# Autodesk Inventor assembly: Stewart-Body-KST215MG
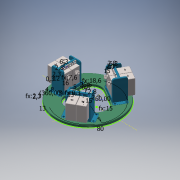
[picture p0: Inventor's stored thumbnail of the model, 180x180]
Saved by Autodesk Inventor 2018.2 (Build 222227000, 227)
## iProperties
Created: 2018-02-25
Part Number: Stewart-Body-KST215MG
Material: Generisch
Document SubType Name: Assembly
Designer: JochenAlt
Author: JochenAlt
## Documents named in this file (6)
- D:\Projects\Donna\CAD\KST DS215MG\Stewart-Body-KST215MG.iam
- D:\Projects\Donna\CAD\KST DS215MG\Stewart-Body.ipt
- D:\Projects\Donna\CAD\KST DS215MG\Stewart-Body-Servo-Holder-KST-DS215.ipt
- Body-Servo-Holder-KST-DS215.ipt
- D:\Projects\Donna\CAD\KST DS215MG\Servo-KST-DS215MG.ipt
- D:\Projects\Donna\CAD\KST DS215MG\Ball-Joint-male.ipt
## Components (16 placed, 4 different names)
1. Stewart-Plate:1 — Passend:1, Passend:2, Passend:3, Passend:4, Passend:5, Passend:10, Passend:11, Passend:16, Passend:17, Passend:22, Passend:23, Passend:24, Passend:25, Passend:26, Passend:27, Passend:28, Passend:29, Passend:30, Passend:31, Passend:32, Passend:33
2. Body-Servo-Holder-KST-DS215:1 — Passend:4, Passend:5, Passend:6, Passend:7, Passend:8, Passend:9
3. Body-Servo-Holder-KST-DS215:2 — Passend:10, Passend:11, Passend:34, Passend:35, Passend:36, Passend:37
4. Body-Servo-Holder-KST-DS215:4 — Passend:16, Passend:17, Passend:18, Passend:19, Passend:20, Passend:21
5. Servo-KST-DS215MG:1 — Passend:6, Passend:7
6. Servo-KST-DS215MG:2 — Passend:8, Passend:9
7. Servo-KST-DS215MG:5 — Passend:20, Passend:21
8. Servo-KST-DS215MG:6 — Passend:18, Passend:19
9. ball joint:1 — Passend:22, Passend:28
10. ball joint:2 — Passend:23, Passend:29
11. ball joint:3 — Passend:24, Passend:33
12. ball joint:4 — Passend:25, Passend:32
13. ball joint:5 — Passend:26, Passend:31
14. ball joint:6 — Passend:27, Passend:30
15. Servo-KST-DS215MG:7 — Passend:34, Passend:36
16. Servo-KST-DS215MG:8 — Passend:35, Passend:37
## Relationships (33: Mate 33)
- Passend:1 [Mate]: Stewart-Plate:1
- Passend:2 [Mate]: Stewart-Plate:1
- Passend:3 [Mate]: Stewart-Plate:1
- Passend:4 [Mate]: Stewart-Plate:1 ↔ Body-Servo-Holder-KST-DS215:1
- Passend:5 [Mate]: Stewart-Plate:1 ↔ Body-Servo-Holder-KST-DS215:1
- Passend:6 [Mate]: Body-Servo-Holder-KST-DS215:1 ↔ Servo-KST-DS215MG:1
- Passend:7 [Mate]: Body-Servo-Holder-KST-DS215:1 ↔ Servo-KST-DS215MG:1
- Passend:8 [Mate]: Body-Servo-Holder-KST-DS215:1 ↔ Servo-KST-DS215MG:2
- Passend:9 [Mate]: Body-Servo-Holder-KST-DS215:1 ↔ Servo-KST-DS215MG:2
- Passend:10 [Mate]: Stewart-Plate:1 ↔ Body-Servo-Holder-KST-DS215:2
- Passend:11 [Mate]: Stewart-Plate:1 ↔ Body-Servo-Holder-KST-DS215:2
- Passend:16 [Mate]: Stewart-Plate:1 ↔ Body-Servo-Holder-KST-DS215:4
- Passend:17 [Mate]: Stewart-Plate:1 ↔ Body-Servo-Holder-KST-DS215:4
- Passend:18 [Mate]: Body-Servo-Holder-KST-DS215:4 ↔ Servo-KST-DS215MG:6
- Passend:19 [Mate]: Body-Servo-Holder-KST-DS215:4 ↔ Servo-KST-DS215MG:6
- Passend:20 [Mate]: Body-Servo-Holder-KST-DS215:4 ↔ Servo-KST-DS215MG:5
- Passend:21 [Mate]: Body-Servo-Holder-KST-DS215:4 ↔ Servo-KST-DS215MG:5
- Passend:22 [Mate]: Stewart-Plate:1 ↔ ball joint:1
- Passend:23 [Mate]: Stewart-Plate:1 ↔ ball joint:2
- Passend:24 [Mate]: Stewart-Plate:1 ↔ ball joint:3
- Passend:25 [Mate]: Stewart-Plate:1 ↔ ball joint:4
- Passend:26 [Mate]: Stewart-Plate:1 ↔ ball joint:5
- Passend:27 [Mate]: Stewart-Plate:1 ↔ ball joint:6
- Passend:28 [Mate]: Stewart-Plate:1 ↔ ball joint:1
- Passend:29 [Mate]: Stewart-Plate:1 ↔ ball joint:2
- Passend:30 [Mate]: Stewart-Plate:1 ↔ ball joint:6
- Passend:31 [Mate]: Stewart-Plate:1 ↔ ball joint:5
- Passend:32 [Mate]: Stewart-Plate:1 ↔ ball joint:4
- Passend:33 [Mate]: Stewart-Plate:1 ↔ ball joint:3
- Passend:34 [Mate]: Body-Servo-Holder-KST-DS215:2 ↔ Servo-KST-DS215MG:7
- Passend:35 [Mate]: Body-Servo-Holder-KST-DS215:2 ↔ Servo-KST-DS215MG:8
- Passend:36 [Mate]: Body-Servo-Holder-KST-DS215:2 ↔ Servo-KST-DS215MG:7
- Passend:37 [Mate]: Body-Servo-Holder-KST-DS215:2 ↔ Servo-KST-DS215MG:8
